# Autodesk Inventor assembly: Grab Articulation axel
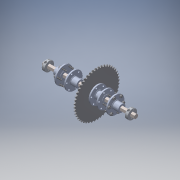
[picture p0: Inventor's stored thumbnail of the model, 180x180]
Saved by Autodesk Inventor 2019 (Build 230136000, 136)
## iProperties
Created: 2019-02-06
Part Number: Grab Articulation axel
Document SubType Name: Assembly
Designer: josh
Author: josh
## Documents named in this file (6)
- D:\Synthesis Robots\Epsilon\Epsilon Grabbers\Grabbing unit\Grab Articulation axel.iam
- D:\Synthesis Robots\Epsilon\Epsilon Grabbers\Grabbing unit\am-0856 500 Hex Shaft for Modulox REV3 - Copy.ipt
- D:\Synthesis Robots\Epsilon\Epsilon Grabbers\Grabbing unit\am-0096a 500 Hex Hub r2.ipt
- D:\Synthesis Robots\Epsilon\Epsilon Grabbers\am-1238 Collar Clamp, 0.5'' Hex Bore, Aluminum REV2.iam
- D:\Synthesis Robots\Epsilon\Epsilon Grabbers\am-0224 48T 35 Chain Bearing Bore Sprocket.ipt
- D:\Synthesis Robots\Epsilon\Swerve drive parts\10-24 Hex Washer Rolling x 3-4_93882A213.ipt
## Components (21 placed, 5 different names)
1. am-0856 500 Hex Shaft for Modulox REV3 - Copy:1
2. am-0096a 500 Hex Hub r2:1
3. am-0096a 500 Hex Hub r2:2
4. am-1238 Collar Clamp, 0.5'' Hex Bore, Aluminum REV2:1 [sub-assembly]
5. am-1238 Collar Clamp, 0.5'' Hex Bore, Aluminum REV2:2 [sub-assembly]
6. am-0096a 500 Hex Hub r2:3
7. am-0096a 500 Hex Hub r2:4
8. am-0096a 500 Hex Hub r2:5
9. am-0224 48T 35 Chain Bearing Bore Sprocket:1
10. 10-24 Hex Washer Rolling x 3-4_93882A213:1
11. 10-24 Hex Washer Rolling x 3-4_93882A213:2
12. 10-24 Hex Washer Rolling x 3-4_93882A213:3
13. 10-24 Hex Washer Rolling x 3-4_93882A213:4
14. 10-24 Hex Washer Rolling x 3-4_93882A213:5
15. 10-24 Hex Washer Rolling x 3-4_93882A213:6
16. 10-24 Hex Washer Rolling x 3-4_93882A213:7
17. 10-24 Hex Washer Rolling x 3-4_93882A213:8
18. 10-24 Hex Washer Rolling x 3-4_93882A213:9
19. 10-24 Hex Washer Rolling x 3-4_93882A213:10
20. 10-24 Hex Washer Rolling x 3-4_93882A213:11
21. 10-24 Hex Washer Rolling x 3-4_93882A213:12
## Relationships (42: Mate 42)
- [Mate]: am-0856 500 Hex Shaft for Modulox REV3 - Copy:1 ↔ am-0096a 500 Hex Hub r2:1
- [Mate]: am-0856 500 Hex Shaft for Modulox REV3 - Copy:1 ↔ am-0096a 500 Hex Hub r2:1
- [Mate]: am-0856 500 Hex Shaft for Modulox REV3 - Copy:1 ↔ am-0096a 500 Hex Hub r2:2
- [Mate]: am-0856 500 Hex Shaft for Modulox REV3 - Copy:1 ↔ am-0096a 500 Hex Hub r2:2
- [Mate]: am-0856 500 Hex Shaft for Modulox REV3 - Copy:1 ↔ am-1238 Collar Clamp, 0.5'' Hex Bore, Aluminum REV2:1
- [Mate]: am-0856 500 Hex Shaft for Modulox REV3 - Copy:1 ↔ am-1238 Collar Clamp, 0.5'' Hex Bore, Aluminum REV2:1
- [Mate]: am-0856 500 Hex Shaft for Modulox REV3 - Copy:1 ↔ am-1238 Collar Clamp, 0.5'' Hex Bore, Aluminum REV2:2
- [Mate]: am-0856 500 Hex Shaft for Modulox REV3 - Copy:1 ↔ am-1238 Collar Clamp, 0.5'' Hex Bore, Aluminum REV2:2
- [Mate]: am-0856 500 Hex Shaft for Modulox REV3 - Copy:1 ↔ am-0096a 500 Hex Hub r2:4
- [Mate]: am-0856 500 Hex Shaft for Modulox REV3 - Copy:1 ↔ am-0096a 500 Hex Hub r2:4
- [Mate]: am-0856 500 Hex Shaft for Modulox REV3 - Copy:1 ↔ am-0096a 500 Hex Hub r2:3
- [Mate]: am-0856 500 Hex Shaft for Modulox REV3 - Copy:1 ↔ am-0096a 500 Hex Hub r2:3
- [Mate]: am-0096a 500 Hex Hub r2:3 ↔ am-0096a 500 Hex Hub r2:5
- [Mate]: am-0856 500 Hex Shaft for Modulox REV3 - Copy:1 ↔ am-0096a 500 Hex Hub r2:5
- [Mate]: am-0856 500 Hex Shaft for Modulox REV3 - Copy:1 ↔ am-0096a 500 Hex Hub r2:5
- [Mate]: am-0096a 500 Hex Hub r2:5 ↔ am-0224 48T 35 Chain Bearing Bore Sprocket:1
- [Mate]: am-0096a 500 Hex Hub r2:5 ↔ am-0224 48T 35 Chain Bearing Bore Sprocket:1
- [Mate]: am-0096a 500 Hex Hub r2:5 ↔ am-0224 48T 35 Chain Bearing Bore Sprocket:1
- [Mate]: am-0096a 500 Hex Hub r2:1 ↔ 10-24 Hex Washer Rolling x 3-4_93882A213:1
- [Mate]: am-0096a 500 Hex Hub r2:1 ↔ 10-24 Hex Washer Rolling x 3-4_93882A213:1
- [Mate]: am-0096a 500 Hex Hub r2:1 ↔ 10-24 Hex Washer Rolling x 3-4_93882A213:6
- [Mate]: am-0096a 500 Hex Hub r2:1 ↔ 10-24 Hex Washer Rolling x 3-4_93882A213:3
- [Mate]: am-0096a 500 Hex Hub r2:1 ↔ 10-24 Hex Washer Rolling x 3-4_93882A213:5
- [Mate]: am-0096a 500 Hex Hub r2:1 ↔ 10-24 Hex Washer Rolling x 3-4_93882A213:4
- [Mate]: am-0096a 500 Hex Hub r2:1 ↔ 10-24 Hex Washer Rolling x 3-4_93882A213:2
- [Mate]: am-0096a 500 Hex Hub r2:1 ↔ 10-24 Hex Washer Rolling x 3-4_93882A213:3
- [Mate]: am-0096a 500 Hex Hub r2:1 ↔ 10-24 Hex Washer Rolling x 3-4_93882A213:5
- [Mate]: am-0096a 500 Hex Hub r2:1 ↔ 10-24 Hex Washer Rolling x 3-4_93882A213:4
- [Mate]: am-0096a 500 Hex Hub r2:1 ↔ 10-24 Hex Washer Rolling x 3-4_93882A213:2
- [Mate]: am-0096a 500 Hex Hub r2:1 ↔ 10-24 Hex Washer Rolling x 3-4_93882A213:6
- [Mate]: am-0096a 500 Hex Hub r2:2 ↔ 10-24 Hex Washer Rolling x 3-4_93882A213:10
- [Mate]: am-0096a 500 Hex Hub r2:2 ↔ 10-24 Hex Washer Rolling x 3-4_93882A213:7
- [Mate]: am-0096a 500 Hex Hub r2:2 ↔ 10-24 Hex Washer Rolling x 3-4_93882A213:11
- [Mate]: am-0096a 500 Hex Hub r2:2 ↔ 10-24 Hex Washer Rolling x 3-4_93882A213:8
- [Mate]: am-0096a 500 Hex Hub r2:2 ↔ 10-24 Hex Washer Rolling x 3-4_93882A213:12
- [Mate]: am-0096a 500 Hex Hub r2:2 ↔ 10-24 Hex Washer Rolling x 3-4_93882A213:9
- [Mate]: am-0096a 500 Hex Hub r2:2 ↔ 10-24 Hex Washer Rolling x 3-4_93882A213:9
- [Mate]: am-0096a 500 Hex Hub r2:2 ↔ 10-24 Hex Washer Rolling x 3-4_93882A213:12
- [Mate]: am-0096a 500 Hex Hub r2:2 ↔ 10-24 Hex Washer Rolling x 3-4_93882A213:11
- [Mate]: am-0096a 500 Hex Hub r2:2 ↔ 10-24 Hex Washer Rolling x 3-4_93882A213:8
- [Mate]: am-0096a 500 Hex Hub r2:2 ↔ 10-24 Hex Washer Rolling x 3-4_93882A213:10
- [Mate]: am-0096a 500 Hex Hub r2:2 ↔ 10-24 Hex Washer Rolling x 3-4_93882A213:7
